# Autodesk Inventor assembly: Inkpath
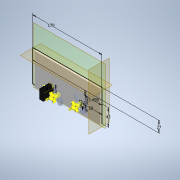
[picture p0: Inventor's stored thumbnail of the model, 180x180]
Saved by Autodesk Inventor 2022 (Build 260153000, 153)
## iProperties
Created: 2024-04-03
Part Number: Inkpath
Document SubType Name: Assembly
Designer: Gotham City
Author: Gotham City
## Documents named in this file (4)
- E:\Xaar128\Inkpath.iam
- E:\Xaar128\Inkpath_Plate.ipt
- E:\Xaar128\Pressuresensor_Holder.ipt
- E:\Xaar128\Dreiwegehahn.ipt
## Components (4 placed, 3 different names)
1. Inkpath_Plate:1 — Flush:1, Flush:2, Flush:3, Mate:1, Angle:1, Flush:4, Flush:5
2. Pressuresensor_Holder:1 — Mate:1, Angle:1, Flush:4, Flush:5
3. Dreiwegehahn:1
4. Dreiwegehahn:2
## Relationships (7: Flush 5, Mate 1, Angle 1)
- Flush:1: Inkpath_Plate:1
- Flush:2: Inkpath_Plate:1
- Flush:3: Inkpath_Plate:1
- Mate:1: Inkpath_Plate:1 ↔ Pressuresensor_Holder:1
- Angle:1 (0 deg): Inkpath_Plate:1 ↔ Pressuresensor_Holder:1
- Flush:4: Inkpath_Plate:1 ↔ Pressuresensor_Holder:1
- Flush:5 (5 mm): Inkpath_Plate:1 ↔ Pressuresensor_Holder:1
